# Autodesk Inventor assembly: openmv_cennt
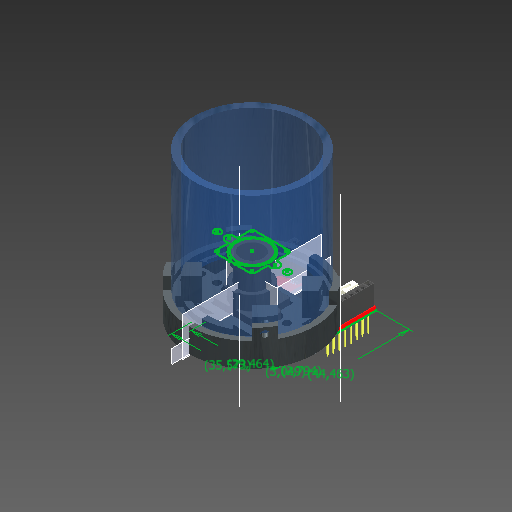
[picture p0: Inventor's stored thumbnail of the model, 512x512]
Saved by Autodesk Inventor 2023 (Build 270158000, 158)
## iProperties
Created: 2025-06-30
Part Number: openmv_cennt
Document SubType Name: Assembly
Designer: daa
Author: daa
## Documents named in this file (4)
- C:\Users\daa\Documents\DASH_V2\openmv_cennt.iam
- C:\Users\daa\Documents\DASH_V2\omv_centre.ipt
- C:\Users\daa\Documents\DASH_V2\openmv h7 plus alt.iam
- C:\Users\daa\Documents\DASH_\Dash-V1\t.ipt
## Components (3 placed, 3 different names)
1. omv_centre:1 — С поворотом:2, С поворотом:3
2. t:1 — С поворотом:2
3. openmv h7 plus alt:1 [sub-assembly] — С поворотом:3
## Relationships (2: RevoluteJoint 2)
- С поворотом:2 [RevoluteJoint]: omv_centre:1 ↔ t:1
- С поворотом:3 [RevoluteJoint] (-1 mm): omv_centre:1 ↔ openmv h7 plus alt:1
